# Autodesk Inventor assembly: Right Door Assembly
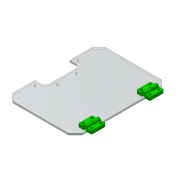
[picture p0: Inventor's stored thumbnail of the model, 180x180]
Saved by Autodesk Inventor 2015 (Build 190159000, 159)
## iProperties
Created: 2018-06-08
Part Number: Right Door Assembly
Document SubType Name: Assembly
Designer: Ghassan Yusuf
Author: Ghassan Yusuf
## Documents named in this file (3)
- X:\Autodesk Designs\MakerBot Transformation\Right Door Assembly.iam
- X:\Autodesk Designs\MakerBot Transformation\Clear Right Side Door.ipt
- X:\Autodesk Designs\MakerBot Transformation\Hing Assambly.iam
## Components (3 placed, 2 different names)
1. Clear Right Side Door:1 — Insert:5, Insert:6, Insert:7, Insert:8
2. Hing Assambly:1 [sub-assembly] — Insert:5, Insert:6, Flush:1
3. Hing Assambly:2 [sub-assembly] — Insert:7, Insert:8, Flush:1
## Relationships (5: Insert 4, Flush 1)
- Insert:5: Clear Right Side Door:1 ↔ Hing Assambly:1
- Insert:6: Clear Right Side Door:1 ↔ Hing Assambly:1
- Insert:7: Clear Right Side Door:1 ↔ Hing Assambly:2
- Insert:8: Clear Right Side Door:1 ↔ Hing Assambly:2
- Flush:1: Hing Assambly:1 ↔ Hing Assambly:2
